# Autodesk Inventor assembly: Assembly
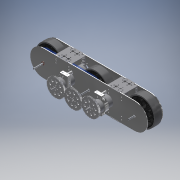
[picture p0: Inventor's stored thumbnail of the model, 180x180]
Saved by Autodesk Inventor 2017 (Build 210142000, 142)
## iProperties
Created: 2017-05-20
Part Number: Assembly
Document SubType Name: Assembly
Designer: steve
Author: steve
## Documents named in this file (18)
- C:\Users\steve\Documents\Inventor\Ultimate FTC Drivebase\Assembly.iam
- C:\Users\steve\Documents\Inventor\Ultimate FTC Drivebase\SidePlate.ipt
- C:\Users\steve\Downloads\am-2648_4inWheel8mmHub.ipt
- C:\Users\steve\Downloads\Tetrix_Kit_FTC\tetrix_739079_collar_2012.ipt
- C:\Users\steve\Downloads\am-2964NeveRest.ipt
- C:\Users\steve\Downloads\Tetrex 2pc motor mount.ipt
- C:\Users\steve\Downloads\Tetrix_Kit_FTC\tetrix_739064_2012.ipt
- C:\Users\steve\Downloads\Tetrix_Kit_FTC\tetrix_739086_2012.ipt
- C:\Users\steve\Downloads\Tetrix_Kit_FTC\tetrix_739088_2012.ipt
- C:\Users\steve\Downloads\Tetrix_Kit_FTC\tetrix_739069_2012.ipt
- C:\Users\steve\Downloads\Tetrix_Kit_FTC\tetrix_739101_2012.ipt
- C:\Users\steve\Downloads\Tetrix_Kit_FTC\tetrix_739097_2012.ipt
- C:\Users\steve\Downloads\Tetrix_Kit_FTC\tetrix_739195_2012.ipt
- C:\Users\steve\Downloads\91831A007_TYPE 18-8 STAINLESS STL NYLON-INSERT LOCKNUT.ipt
- C:\Users\steve\Downloads\am-3284+32tNinjaStarSprocket.ipt
- C:\Users\steve\Documents\Inventor\Ultimate FTC Drivebase\Assembly\Design Accelerator\Chain Drive3.iam
- C:\Users\steve\Documents\Inventor\Ultimate FTC Drivebase\Assembly\Design Accelerator\Chain Drive4.iam
- C:\Users\steve\Downloads\Tetrix_Kit_FTC\tetrix_739091_2012.ipt
## Components (79 placed, 16 different names)
1. SidePlate:1 — Mate:1, Mate:2, Mate:3, Flush:1, Mate:8, Mate:9, Mate:15, Mate:16, Flush:4, Flush:5, Mate:25, Mate:27, Mate:47, Mate:48, Mate:67, Mate:68, Mate:69, Mate:70, Mate:71, Mate:72, Mate:73, Mate:74, Mate:86, Mate:88, Mate:90, Mate:92, Mate:145, Mate:146, Mate:147, Mate:149, Mate:150, Mate:151, Mate:152, Mate:153, Mate:154, Mate:155, Mate:156, Mate:157, Mate:158, Mate:181, Mate:182
2. am-2648_4inWheel8mmHub:1 — Mate:3, Mate:11
3. am-2648_4inWheel8mmHub:2 — Mate:2, Mate:14
4. am-2648_4inWheel8mmHub:3 — Mate:1
5. SidePlate:2 — Flush:1, Mate:8, Mate:15, Mate:17, Mate:18, Mate:19, Angle:1, Angle:2, Mate:33, Mate:35, Mate:36, Mate:37, Flush:29, Mate:45, Mate:50, Mate:62, Mate:66, Mate:94, Mate:106, Mate:107, Mate:108, Mate:109, Mate:110, Mate:111, Mate:112, Mate:113, Mate:114, Mate:148, Mate:159, Mate:160, Mate:161, Mate:162, Mate:163, Mate:164, Mate:165, Mate:166, Mate:184
6. tetrix_739079_collar_2012:1 — Mate:9, Mate:11, Mate:143
7. tetrix_739079_collar_2012:2 — Mate:14, Mate:144
8. am-2964NeveRest:1 — Mate:19, Flush:5, Mate:21, Mate:34
9. am-2964NeveRest:2 — Mate:18, Flush:4, Mate:20, Mate:32
10. Tetrex 2pc motor mount:1 — Mate:21, Angle:1, Mate:49, Mate:53, Mate:56, Mate:57
11. Tetrex 2pc motor mount:2 — Mate:20, Angle:2, Mate:60, Mate:61, Mate:65, Mate:83, Mate:84, Mate:103, Mate:104
12. tetrix_739064_2012:1 — Mate:27, Mate:42, Mate:43, Symmetry:2, Mate:48, Mate:127, Mate:128, Mate:129, Mate:130
13. tetrix_739064_2012:2 — Mate:25, Symmetry:2, Mate:46, Mate:47
14. tetrix_739086_2012:1 — Mate:32, Tangent:2, Flush:28
15. tetrix_739086_2012:2 — Mate:33, Tangent:1, Tangent:2, Flush:27, Flush:28
16. tetrix_739086_2012:3 — Mate:34, Tangent:1, Flush:27
17. tetrix_739088_2012:1 — Mate:37, Mate:139
18. tetrix_739088_2012:2 — Mate:35, Mate:141, Mate:183
19. tetrix_739088_2012:3 — Mate:36, Mate:140, Mate:142
20. tetrix_739069_2012:1
21. tetrix_739069_2012:2 — Mate:42, Mate:43, Mate:46
22. tetrix_739101_2012:1 — Mate:49, Mate:50, Mate:51, Mate:52
23. tetrix_739101_2012:2 — Mate:51, Mate:52, Mate:53
24. tetrix_739101_2012:3 — Mate:54, Mate:55, Mate:56, Mate:57
25. tetrix_739101_2012:4 — Mate:54, Mate:55
26. tetrix_739101_2012:5 — Mate:63, Mate:64, Mate:66
27. tetrix_739101_2012:6 — Mate:63, Mate:64, Mate:65
28. tetrix_739101_2012:7 — Mate:58, Mate:59, Mate:60, Mate:61
29. tetrix_739101_2012:8 — Mate:58, Mate:59, Mate:62
30. tetrix_739097_2012:1 — Mate:73, Mate:74, Mate:91
31. tetrix_739097_2012:2 — Mate:67, Mate:68, Mate:85
32. tetrix_739097_2012:3 — Mate:69, Mate:70, Mate:87
33. tetrix_739097_2012:4 — Mate:71, Mate:72, Mate:89
34. tetrix_739195_2012:1 — Mate:83, Mate:84, Mate:93
35. 91831A007_TYPE 18-8 STAINLESS STL NYLON-INSERT LOCKNUT:1 — Mate:89, Mate:90
36. 91831A007_TYPE 18-8 STAINLESS STL NYLON-INSERT LOCKNUT:2 — Mate:91, Mate:92
37. 91831A007_TYPE 18-8 STAINLESS STL NYLON-INSERT LOCKNUT:3 — Mate:87, Mate:88
38. 91831A007_TYPE 18-8 STAINLESS STL NYLON-INSERT LOCKNUT:4 — Mate:85, Mate:86
39. 91831A007_TYPE 18-8 STAINLESS STL NYLON-INSERT LOCKNUT:5 — Mate:93, Mate:94
40. tetrix_739195_2012:2 — Mate:103, Mate:104, Mate:105
41. 91831A007_TYPE 18-8 STAINLESS STL NYLON-INSERT LOCKNUT:10 — Mate:105, Mate:106
42. tetrix_739097_2012:9 — Mate:107, Mate:108, Mate:123
43. tetrix_739097_2012:10 — Mate:109, Mate:110, Mate:126
44. tetrix_739097_2012:11 — Mate:113, Mate:114, Mate:125
45. tetrix_739097_2012:12 — Mate:111, Mate:112, Mate:124
46. 91831A007_TYPE 18-8 STAINLESS STL NYLON-INSERT LOCKNUT:11 — Mate:125, Mate:128
47. 91831A007_TYPE 18-8 STAINLESS STL NYLON-INSERT LOCKNUT:12
48. 91831A007_TYPE 18-8 STAINLESS STL NYLON-INSERT LOCKNUT:13
49. 91831A007_TYPE 18-8 STAINLESS STL NYLON-INSERT LOCKNUT:14 — Mate:123, Mate:129
50. 91831A007_TYPE 18-8 STAINLESS STL NYLON-INSERT LOCKNUT:15
51. 91831A007_TYPE 18-8 STAINLESS STL NYLON-INSERT LOCKNUT:16 — Mate:124, Mate:130
52. 91831A007_TYPE 18-8 STAINLESS STL NYLON-INSERT LOCKNUT:17
53. 91831A007_TYPE 18-8 STAINLESS STL NYLON-INSERT LOCKNUT:18 — Mate:126, Mate:127
54. am-3284+32tNinjaStarSprocket:1 — Mate:141, Flush:30, Mate:143
55. am-3284+32tNinjaStarSprocket:2 — Mate:142, Flush:30, Mate:144
56. am-3284+32tNinjaStarSprocket:3 — Mate:139, Flush:31
57. am-3284+32tNinjaStarSprocket:4 — Mate:140, Flush:31
58. Chain Drive:1 [sub-assembly]
59. Chain Drive:2 [sub-assembly]
60. tetrix_739064_2012:3 — Mate:148, Mate:149, Mate:150, Mate:171, Mate:172, Mate:173, Mate:174, Mate:179, Mate:180
61. tetrix_739064_2012:4 — Mate:145, Mate:146, Mate:147
62. tetrix_739097_2012:13 — Mate:155, Mate:156, Mate:169
63. tetrix_739097_2012:14 — Mate:151, Mate:152, Mate:168
64. tetrix_739097_2012:15 — Mate:157, Mate:158, Mate:170
65. tetrix_739097_2012:16 — Mate:153, Mate:154, Mate:167
66. tetrix_739097_2012:17 — Mate:162, Mate:164, Mate:178
67. tetrix_739097_2012:18 — Mate:161, Mate:165, Mate:176
68. tetrix_739097_2012:19 — Mate:160, Mate:166, Mate:175
69. tetrix_739097_2012:20 — Mate:159, Mate:163, Mate:177
70. 91831A007_TYPE 18-8 STAINLESS STL NYLON-INSERT LOCKNUT:19 — Mate:167, Mate:173
71. 91831A007_TYPE 18-8 STAINLESS STL NYLON-INSERT LOCKNUT:20 — Mate:169, Mate:172
72. 91831A007_TYPE 18-8 STAINLESS STL NYLON-INSERT LOCKNUT:21 — Mate:170, Mate:171
73. 91831A007_TYPE 18-8 STAINLESS STL NYLON-INSERT LOCKNUT:22 — Mate:168, Mate:174
74. 91831A007_TYPE 18-8 STAINLESS STL NYLON-INSERT LOCKNUT:23 — Mate:176, Mate:180
75. 91831A007_TYPE 18-8 STAINLESS STL NYLON-INSERT LOCKNUT:24 — Mate:178
76. 91831A007_TYPE 18-8 STAINLESS STL NYLON-INSERT LOCKNUT:25 — Mate:177
77. 91831A007_TYPE 18-8 STAINLESS STL NYLON-INSERT LOCKNUT:26 — Mate:175, Mate:179
78. tetrix_739091_2012:1 — Mate:181, Mate:182
79. tetrix_739091_2012:2 — Mate:183, Mate:184
## Relationships (145: Mate 132, Flush 8, Angle 2, Tangent 2, Symmetry 1)
- Mate:1: SidePlate:1 ↔ am-2648_4inWheel8mmHub:3
- Mate:2: SidePlate:1 ↔ am-2648_4inWheel8mmHub:2
- Mate:3: SidePlate:1 ↔ am-2648_4inWheel8mmHub:1
- Flush:1: SidePlate:1 ↔ SidePlate:2
- Mate:8 (53.2 mm): SidePlate:1 ↔ SidePlate:2
- Mate:9: SidePlate:1 ↔ tetrix_739079_collar_2012:1
- Mate:11: am-2648_4inWheel8mmHub:1 ↔ tetrix_739079_collar_2012:1
- Mate:14: am-2648_4inWheel8mmHub:2 ↔ tetrix_739079_collar_2012:2
- Mate:15: SidePlate:1 ↔ SidePlate:2
- Mate:16: SidePlate:1
- Mate:17: SidePlate:2
- Mate:18: SidePlate:2 ↔ am-2964NeveRest:2
- Mate:19: SidePlate:2 ↔ am-2964NeveRest:1
- Flush:4: SidePlate:1 ↔ am-2964NeveRest:2
- Flush:5: SidePlate:1 ↔ am-2964NeveRest:1
- Mate:20: am-2964NeveRest:2 ↔ Tetrex 2pc motor mount:2
- Mate:21: am-2964NeveRest:1 ↔ Tetrex 2pc motor mount:1
- Angle:1 (0 deg): SidePlate:2 ↔ Tetrex 2pc motor mount:1
- Angle:2 (0 deg): SidePlate:2 ↔ Tetrex 2pc motor mount:2
- Mate:25: SidePlate:1 ↔ tetrix_739064_2012:2
- Mate:27: SidePlate:1 ↔ tetrix_739064_2012:1
- Mate:32: am-2964NeveRest:2 ↔ tetrix_739086_2012:1
- Mate:33: SidePlate:2 ↔ tetrix_739086_2012:2
- Mate:34: am-2964NeveRest:1 ↔ tetrix_739086_2012:3
- Tangent:1: tetrix_739086_2012:2 ↔ tetrix_739086_2012:3
- Tangent:2: tetrix_739086_2012:1 ↔ tetrix_739086_2012:2
- Flush:27: tetrix_739086_2012:2 ↔ tetrix_739086_2012:3
- Flush:28: tetrix_739086_2012:1 ↔ tetrix_739086_2012:2
- Mate:35: SidePlate:2 ↔ tetrix_739088_2012:2
- Mate:36: SidePlate:2 ↔ tetrix_739088_2012:3
- Mate:37: SidePlate:2 ↔ tetrix_739088_2012:1
- Flush:29: SidePlate:2
- Mate:42: tetrix_739064_2012:1 ↔ tetrix_739069_2012:2
- Mate:43: tetrix_739064_2012:1 ↔ tetrix_739069_2012:2
- Symmetry:2: tetrix_739064_2012:1 ↔ tetrix_739064_2012:2
- Mate:45: SidePlate:2
- Mate:46: tetrix_739064_2012:2 ↔ tetrix_739069_2012:2
- Mate:47: SidePlate:1 ↔ tetrix_739064_2012:2
- Mate:48: SidePlate:1 ↔ tetrix_739064_2012:1
- Mate:49: Tetrex 2pc motor mount:1 ↔ tetrix_739101_2012:1
- Mate:50: SidePlate:2 ↔ tetrix_739101_2012:1
- Mate:51: tetrix_739101_2012:1 ↔ tetrix_739101_2012:2
- Mate:52: tetrix_739101_2012:1 ↔ tetrix_739101_2012:2
- Mate:53: Tetrex 2pc motor mount:1 ↔ tetrix_739101_2012:2
- Mate:54: tetrix_739101_2012:3 ↔ tetrix_739101_2012:4
- Mate:55: tetrix_739101_2012:3 ↔ tetrix_739101_2012:4
- Mate:56: Tetrex 2pc motor mount:1 ↔ tetrix_739101_2012:3
- Mate:57: Tetrex 2pc motor mount:1 ↔ tetrix_739101_2012:3
- Mate:58: tetrix_739101_2012:7 ↔ tetrix_739101_2012:8
- Mate:59: tetrix_739101_2012:7 ↔ tetrix_739101_2012:8
- Mate:60: Tetrex 2pc motor mount:2 ↔ tetrix_739101_2012:7
- Mate:61: Tetrex 2pc motor mount:2 ↔ tetrix_739101_2012:7
- Mate:62: SidePlate:2 ↔ tetrix_739101_2012:8
- Mate:63: tetrix_739101_2012:5 ↔ tetrix_739101_2012:6
- Mate:64: tetrix_739101_2012:5 ↔ tetrix_739101_2012:6
- Mate:65: Tetrex 2pc motor mount:2 ↔ tetrix_739101_2012:6
- Mate:66: SidePlate:2 ↔ tetrix_739101_2012:5
- Mate:67: SidePlate:1 ↔ tetrix_739097_2012:2
- Mate:68: SidePlate:1 ↔ tetrix_739097_2012:2
- Mate:69: SidePlate:1 ↔ tetrix_739097_2012:3
- Mate:70: SidePlate:1 ↔ tetrix_739097_2012:3
- Mate:71: SidePlate:1 ↔ tetrix_739097_2012:4
- Mate:72: SidePlate:1 ↔ tetrix_739097_2012:4
- Mate:73: SidePlate:1 ↔ tetrix_739097_2012:1
- Mate:74: SidePlate:1 ↔ tetrix_739097_2012:1
- Mate:83: Tetrex 2pc motor mount:2 ↔ tetrix_739195_2012:1
- Mate:84: Tetrex 2pc motor mount:2 ↔ tetrix_739195_2012:1
- Mate:85: tetrix_739097_2012:2 ↔ 91831A007_TYPE 18-8 STAINLESS STL NYLON-INSERT LOCKNUT:4
- Mate:86: SidePlate:1 ↔ 91831A007_TYPE 18-8 STAINLESS STL NYLON-INSERT LOCKNUT:4
- Mate:87: tetrix_739097_2012:3 ↔ 91831A007_TYPE 18-8 STAINLESS STL NYLON-INSERT LOCKNUT:3
- Mate:88: SidePlate:1 ↔ 91831A007_TYPE 18-8 STAINLESS STL NYLON-INSERT LOCKNUT:3
- Mate:89: tetrix_739097_2012:4 ↔ 91831A007_TYPE 18-8 STAINLESS STL NYLON-INSERT LOCKNUT:1
- Mate:90: SidePlate:1 ↔ 91831A007_TYPE 18-8 STAINLESS STL NYLON-INSERT LOCKNUT:1
- Mate:91: tetrix_739097_2012:1 ↔ 91831A007_TYPE 18-8 STAINLESS STL NYLON-INSERT LOCKNUT:2
- Mate:92: SidePlate:1 ↔ 91831A007_TYPE 18-8 STAINLESS STL NYLON-INSERT LOCKNUT:2
- Mate:93: tetrix_739195_2012:1 ↔ 91831A007_TYPE 18-8 STAINLESS STL NYLON-INSERT LOCKNUT:5
- Mate:94: SidePlate:2 ↔ 91831A007_TYPE 18-8 STAINLESS STL NYLON-INSERT LOCKNUT:5
- Mate:103: Tetrex 2pc motor mount:2 ↔ tetrix_739195_2012:2
- Mate:104: Tetrex 2pc motor mount:2 ↔ tetrix_739195_2012:2
- Mate:105: tetrix_739195_2012:2 ↔ 91831A007_TYPE 18-8 STAINLESS STL NYLON-INSERT LOCKNUT:10
- Mate:106: SidePlate:2 ↔ 91831A007_TYPE 18-8 STAINLESS STL NYLON-INSERT LOCKNUT:10
- Mate:107: SidePlate:2 ↔ tetrix_739097_2012:9
- Mate:108: SidePlate:2 ↔ tetrix_739097_2012:9
- Mate:109: SidePlate:2 ↔ tetrix_739097_2012:10
- Mate:110: SidePlate:2 ↔ tetrix_739097_2012:10
- Mate:111: SidePlate:2 ↔ tetrix_739097_2012:12
- Mate:112: SidePlate:2 ↔ tetrix_739097_2012:12
- Mate:113: SidePlate:2 ↔ tetrix_739097_2012:11
- Mate:114: SidePlate:2 ↔ tetrix_739097_2012:11
- Mate:123: tetrix_739097_2012:9 ↔ 91831A007_TYPE 18-8 STAINLESS STL NYLON-INSERT LOCKNUT:14
- Mate:124: tetrix_739097_2012:12 ↔ 91831A007_TYPE 18-8 STAINLESS STL NYLON-INSERT LOCKNUT:16
- Mate:125: tetrix_739097_2012:11 ↔ 91831A007_TYPE 18-8 STAINLESS STL NYLON-INSERT LOCKNUT:11
- Mate:126: tetrix_739097_2012:10 ↔ 91831A007_TYPE 18-8 STAINLESS STL NYLON-INSERT LOCKNUT:18
- Mate:127: tetrix_739064_2012:1 ↔ 91831A007_TYPE 18-8 STAINLESS STL NYLON-INSERT LOCKNUT:18
- Mate:128: tetrix_739064_2012:1 ↔ 91831A007_TYPE 18-8 STAINLESS STL NYLON-INSERT LOCKNUT:11
- Mate:129: tetrix_739064_2012:1 ↔ 91831A007_TYPE 18-8 STAINLESS STL NYLON-INSERT LOCKNUT:14
- Mate:130: tetrix_739064_2012:1 ↔ 91831A007_TYPE 18-8 STAINLESS STL NYLON-INSERT LOCKNUT:16
- Mate:139: tetrix_739088_2012:1 ↔ am-3284+32tNinjaStarSprocket:3
- Mate:140: tetrix_739088_2012:3 ↔ am-3284+32tNinjaStarSprocket:4
- Mate:141: tetrix_739088_2012:2 ↔ am-3284+32tNinjaStarSprocket:1
- Mate:142: tetrix_739088_2012:3 ↔ am-3284+32tNinjaStarSprocket:2
- Flush:30: am-3284+32tNinjaStarSprocket:1 ↔ am-3284+32tNinjaStarSprocket:2
- Flush:31: am-3284+32tNinjaStarSprocket:3 ↔ am-3284+32tNinjaStarSprocket:4
- Mate:143: tetrix_739079_collar_2012:1 ↔ am-3284+32tNinjaStarSprocket:1
- Mate:144: tetrix_739079_collar_2012:2 ↔ am-3284+32tNinjaStarSprocket:2
- Mate:145: SidePlate:1 ↔ tetrix_739064_2012:4
- Mate:146: SidePlate:1 ↔ tetrix_739064_2012:4
- Mate:147: SidePlate:1 ↔ tetrix_739064_2012:4
- Mate:148: SidePlate:2 ↔ tetrix_739064_2012:3
- Mate:149: SidePlate:1 ↔ tetrix_739064_2012:3
- Mate:150: SidePlate:1 ↔ tetrix_739064_2012:3
- Mate:151: SidePlate:1 ↔ tetrix_739097_2012:14
- Mate:152: SidePlate:1 ↔ tetrix_739097_2012:14
- Mate:153: SidePlate:1 ↔ tetrix_739097_2012:16
- Mate:154: SidePlate:1 ↔ tetrix_739097_2012:16
- Mate:155: SidePlate:1 ↔ tetrix_739097_2012:13
- Mate:156: SidePlate:1 ↔ tetrix_739097_2012:13
- Mate:157: SidePlate:1 ↔ tetrix_739097_2012:15
- Mate:158: SidePlate:1 ↔ tetrix_739097_2012:15
- Mate:159: SidePlate:2 ↔ tetrix_739097_2012:20
- Mate:160: SidePlate:2 ↔ tetrix_739097_2012:19
- Mate:161: SidePlate:2 ↔ tetrix_739097_2012:18
- Mate:162: SidePlate:2 ↔ tetrix_739097_2012:17
- Mate:163: SidePlate:2 ↔ tetrix_739097_2012:20
- Mate:164: SidePlate:2 ↔ tetrix_739097_2012:17
- Mate:165: SidePlate:2 ↔ tetrix_739097_2012:18
- Mate:166: SidePlate:2 ↔ tetrix_739097_2012:19
- Mate:167: tetrix_739097_2012:16 ↔ 91831A007_TYPE 18-8 STAINLESS STL NYLON-INSERT LOCKNUT:19
- Mate:168: tetrix_739097_2012:14 ↔ 91831A007_TYPE 18-8 STAINLESS STL NYLON-INSERT LOCKNUT:22
- Mate:169: tetrix_739097_2012:13 ↔ 91831A007_TYPE 18-8 STAINLESS STL NYLON-INSERT LOCKNUT:20
- Mate:170: tetrix_739097_2012:15 ↔ 91831A007_TYPE 18-8 STAINLESS STL NYLON-INSERT LOCKNUT:21
- Mate:171: tetrix_739064_2012:3 ↔ 91831A007_TYPE 18-8 STAINLESS STL NYLON-INSERT LOCKNUT:21
- Mate:172: tetrix_739064_2012:3 ↔ 91831A007_TYPE 18-8 STAINLESS STL NYLON-INSERT LOCKNUT:20
- Mate:173: tetrix_739064_2012:3 ↔ 91831A007_TYPE 18-8 STAINLESS STL NYLON-INSERT LOCKNUT:19
- Mate:174: tetrix_739064_2012:3 ↔ 91831A007_TYPE 18-8 STAINLESS STL NYLON-INSERT LOCKNUT:22
- Mate:175: tetrix_739097_2012:19 ↔ 91831A007_TYPE 18-8 STAINLESS STL NYLON-INSERT LOCKNUT:26
- Mate:176: tetrix_739097_2012:18 ↔ 91831A007_TYPE 18-8 STAINLESS STL NYLON-INSERT LOCKNUT:23
- Mate:177: tetrix_739097_2012:20 ↔ 91831A007_TYPE 18-8 STAINLESS STL NYLON-INSERT LOCKNUT:25
- Mate:178: tetrix_739097_2012:17 ↔ 91831A007_TYPE 18-8 STAINLESS STL NYLON-INSERT LOCKNUT:24
- Mate:179: tetrix_739064_2012:3 ↔ 91831A007_TYPE 18-8 STAINLESS STL NYLON-INSERT LOCKNUT:26
- Mate:180: tetrix_739064_2012:3 ↔ 91831A007_TYPE 18-8 STAINLESS STL NYLON-INSERT LOCKNUT:23
- Mate:181: SidePlate:1 ↔ tetrix_739091_2012:1
- Mate:182: SidePlate:1 ↔ tetrix_739091_2012:1
- Mate:183: tetrix_739088_2012:2 ↔ tetrix_739091_2012:2
- Mate:184: SidePlate:2 ↔ tetrix_739091_2012:2
